# Autodesk Inventor assembly: RCUv2-3Assy
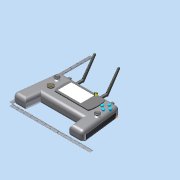
[picture p0: Inventor's stored thumbnail of the model, 180x180]
Saved by Autodesk Inventor 2011 SP1 (Build 150282100, 282)
## iProperties
Created: 2011-08-15
Part Number: RCUv2-3Assy
Document SubType Name: Assembly
Designer: dgitz
Author: dgitz
## Documents named in this file (9)
- C:\Dropbox\ICARUS\Remote Control Unit (RCU)\RCU v2\Design\RCUv2-3Assy.iam
- C:\Dropbox\ICARUS\Remote Control Unit (RCU)\RCU v2\Design\Library\SpringSamsungGalaxySAssy.iam
- C:\Dropbox\ICARUS\Remote Control Unit (RCU)\RCU v2\Design\RCUv2-3\RCUAssy.iam
- C:\Dropbox\ICARUS\Remote Control Unit (RCU)\RCU v2\Design\Imported Components\User Library-Joystick_Asm_Left\Assembly4.iam
- C:\Dropbox\ICARUS\Remote Control Unit (RCU)\RCU v2\Design\Library\XBox360DirectionalPad.ipt
- C:\Dropbox\ICARUS\Remote Control Unit (RCU)\RCU v2\Design\Library\Xbox360Button.ipt
- C:\Dropbox\ICARUS\Remote Control Unit (RCU)\RCU v2\Design\Imported Components\User Library-12 inch scale\Part6.ipt
- C:\Dropbox\ICARUS\Remote Control Unit (RCU)\RCU v2\Design\Imported Components\User Library-12 inch scale\Part8.ipt
- C:\Dropbox\ICARUS\Remote Control Unit (RCU)\RCU v2\Design\RCUv2-3\Grip.ipt
## Components (12 placed, 8 different names)
1. SpringSamsungGalaxySAssy:1 [sub-assembly] — Mate:2, Flush:2
2. RCUAssy:1 [sub-assembly] — Flush:1, Mate:1, Mate:2, Flush:2, Mate:3, Mate:5, Mate:6, Flush:6, Mate:12, Mate:13, Mate:16, Mate:17, Mate:18
3. Assembly4:1 [sub-assembly] — Mate:5
4. Assembly4:2 [sub-assembly] — Mate:6
5. XBox360DirectionalPad:1 — Mate:3, Mate:4
6. Xbox360Button:1 — Flush:5, Mate:7, Mate:10, Mate:11
7. Xbox360Button:2 — Flush:3, Flush:4, Mate:8, Mate:9, Mate:11
8. Xbox360Button:3 — Flush:3, Flush:6, Mate:7, Mate:9
9. Xbox360Button:4 — Flush:4, Flush:5, Mate:8, Mate:10
10. Part6:1 — Flush:7, Mate:12, Mate:13, Mate:14, Flush:8, Mate:15
11. Part8:1 — Mate:14, Flush:8, Mate:15
12. Grip:1 — Mate:16, Mate:17, Mate:18
## Relationships (26: Mate 18, Flush 8)
- Flush:1: RCUAssy:1
- Mate:1: RCUAssy:1
- Mate:2 (-12.7 mm): SpringSamsungGalaxySAssy:1 ↔ RCUAssy:1
- Flush:2 (12.7 mm): SpringSamsungGalaxySAssy:1 ↔ RCUAssy:1
- Mate:3 (-2.54 mm): RCUAssy:1 ↔ XBox360DirectionalPad:1
- Mate:4 (-12.7 mm): XBox360DirectionalPad:1
- Mate:5 (-5.08 mm): RCUAssy:1 ↔ Assembly4:1
- Mate:6 (-5.08 mm): RCUAssy:1 ↔ Assembly4:2
- Flush:3: Xbox360Button:2 ↔ Xbox360Button:3
- Flush:4: Xbox360Button:2 ↔ Xbox360Button:4
- Flush:5: Xbox360Button:1 ↔ Xbox360Button:4
- Flush:6 (-5.08 mm): RCUAssy:1 ↔ Xbox360Button:3
- Mate:7 (19.05 mm): Xbox360Button:1 ↔ Xbox360Button:3
- Mate:8 (19.05 mm): Xbox360Button:2 ↔ Xbox360Button:4
- Mate:9 (19.05 mm): Xbox360Button:2 ↔ Xbox360Button:3
- Mate:10 (19.05 mm): Xbox360Button:1 ↔ Xbox360Button:4
- Mate:11 (26.924 mm): Xbox360Button:1 ↔ Xbox360Button:2
- Flush:7 (38.1 mm): Part6:1
- Mate:12: RCUAssy:1 ↔ Part6:1
- Mate:13: RCUAssy:1 ↔ Part6:1
- Mate:14: Part6:1 ↔ Part8:1
- Flush:8: Part6:1 ↔ Part8:1
- Mate:15: Part6:1 ↔ Part8:1
- Mate:16: RCUAssy:1 ↔ Grip:1
- Mate:17: RCUAssy:1 ↔ Grip:1
- Mate:18 (12.7 mm): RCUAssy:1 ↔ Grip:1
